# Autodesk Inventor assembly: Sample Holder
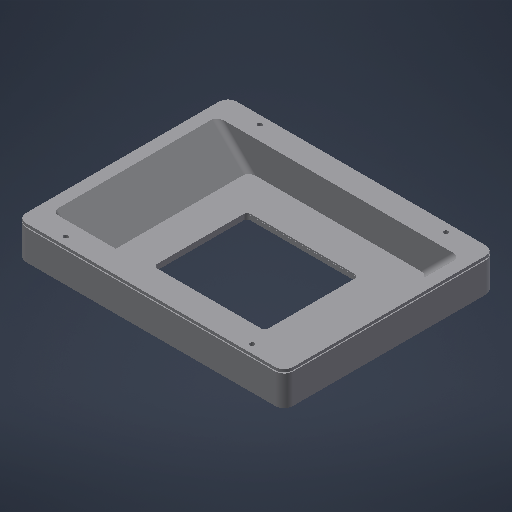
[picture p0: Inventor's stored thumbnail of the model, 512x512]
Saved by Autodesk Inventor 2026 (Build 300175000, 175)
## iProperties
Created: 2026-03-11
Part Number: Sample Holder
Document SubType Name: Assembly
Designer: FiolkaLab
Author: FiolkaLab
## Documents named in this file (3)
- E:\Muaaz\Baseplate\ASLM_DvOPM System Assembly\Sample Holder.iam
- E:\Muaaz\Baseplate\ASLM_DvOPM System Assembly\i-4023-Tai-CoverTop-V3.ipt
- E:\Muaaz\Baseplate\ASLM_DvOPM System Assembly\i-4023-Tai-Base-V3 - Copy.ipt
## Components (2 placed, 2 different names)
1. i-4023-Tai-CoverTop-V3:1 — Mate:1, Mate:2
2. i-4023-Tai-Base-V3 - Copy:1 — Mate:1, Mate:2
## Relationships (2: Mate 2)
- Mate:1: i-4023-Tai-CoverTop-V3:1 ↔ i-4023-Tai-Base-V3 - Copy:1
- Mate:2: i-4023-Tai-CoverTop-V3:1 ↔ i-4023-Tai-Base-V3 - Copy:1
